# Autodesk Inventor assembly: 1Sborka antenn
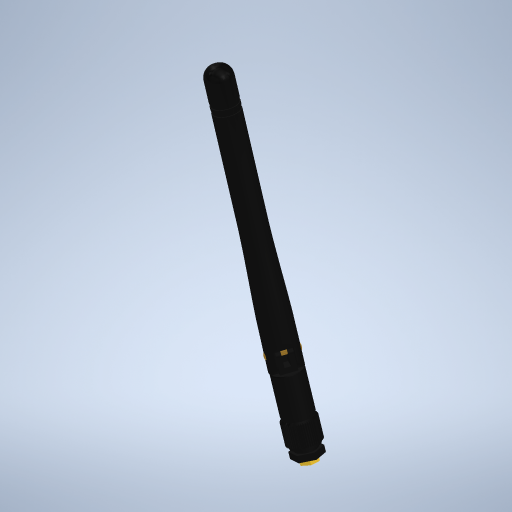
[picture p0: Inventor's stored thumbnail of the model, 512x512]
Saved by Autodesk Inventor 2024 (Build 280153000, 153)
## iProperties
Created: 2023-11-30
Part Number: 1Sborka antenn
Description: STEP AP214
Document SubType Name: Assembly
Designer: Roman Suk
Sending System: SolidWorks 2020
Preprocessor: SwSTEP 2.0
Title: 1Sborka antenn.STEP
Author: admin
Revision Number: ANY
## Documents named in this file (6)
- C:\Users\s21suk\Desktop\Final1\1assemble antenn\1assemble antenn.iam
- C:\Users\s21suk\Desktop\Final1\1assemble antenn\antenn2.ipt
- C:\Users\s21suk\Desktop\Final1\1assemble antenn\antenn1.ipt
- C:\Users\s21suk\Desktop\Final1\1assemble antenn\part3.ipt
- C:\Users\s21suk\Desktop\Final1\1assemble antenn\part4.ipt
- C:\Users\s21suk\Desktop\Final1\1assemble antenn\taper pin unhardened_iso_ISO 2339 - A - 2 x 10 - St.ipt
## Components (5 placed, 5 different names)
1. antenn2_1 — Rotační:2, Vložit:1, Vložit:2
2. antenn1_2 — Rotační:1, Rotační:2
3. part3_3 — Vložit:2
4. part4_4 — Vložit:1
5. taper pin unhardened_iso_ISO 2339 - A - 2 x 10 - St_5 — Rotační:1
## Relationships (4: RevoluteJoint 2, Insert 2)
- Rotační:1 [RevoluteJoint]: antenn1_2 ↔ taper pin unhardened_iso_ISO 2339 - A - 2 x 10 - St_5
- Rotační:2 [RevoluteJoint]: antenn2_1 ↔ antenn1_2
- Vložit:1 [Insert]: antenn2_1 ↔ part4_4
- Vložit:2 [Insert]: antenn2_1 ↔ part3_3
